# Autodesk Inventor assembly: fc16-071
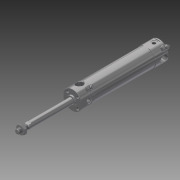
[picture p0: Inventor's stored thumbnail of the model, 180x180]
Saved by Autodesk Inventor 2016 SP1 (Build 200210100, 210)
## iProperties
Category: Pneumatics
Company: Autodesk Inc.
Created: 2015-12-03
Part Number: fc16-071
Catalog Web Link: https://www.phdinc.com/product/?product=cylinders&series=ocg
Document SubType Name: Assembly
Designer: Autodesk Inc.
Vendor: PHD Inc.
Author: Autodesk Inc.
Keywords: FIRSTChoice
## Documents named in this file (6)
- D:\FIRST\FRC KOP 2016\FRC FIRSTChoice 2016\fc16-071_PneuCylinder.iam
- D:\FIRST\FRC KOP 2016\FRC FIRSTChoice 2016\Parts\TUBE_OCG13_4x2_Open-Extend_.ipt
- D:\FIRST\FRC KOP 2016\FRC FIRSTChoice 2016\Parts\HD_OCG13_4x2_Open-Extend.ipt
- D:\FIRST\FRC KOP 2016\FRC FIRSTChoice 2016\Parts\PR_OCG1-3_4x2.ipt
- D:\FIRST\FRC KOP 2016\FRC FIRSTChoice 2016\Parts\PN1972-015_NUT1_4-28-UNF.ipt
- D:\FIRST\FRC KOP 2016\FRC FIRSTChoice 2016\Parts\CAP_OCG1-3_4.ipt
## Components (5 placed, 5 different names)
1. TUBE_OCG13_4x2_Open-Extend_:1 — Insert:1
2. HD_OCG13_4x2_Open-Extend:1 — Angle:1
3. PR_OCG1-3_4x2:1
4. PN1972-015_NUT1_4-28-UNF:1
5. CAP_OCG1-3_4:1 — Insert:1, Angle:1
## Relationships (2: Insert 1, Angle 1)
- Insert:1: TUBE_OCG13_4x2_Open-Extend_:1 ↔ CAP_OCG1-3_4:1
- Angle:1 (0 deg): HD_OCG13_4x2_Open-Extend:1 ↔ CAP_OCG1-3_4:1
